# Autodesk Inventor assembly: ASM_Quarter_Piece_Assembly_Final
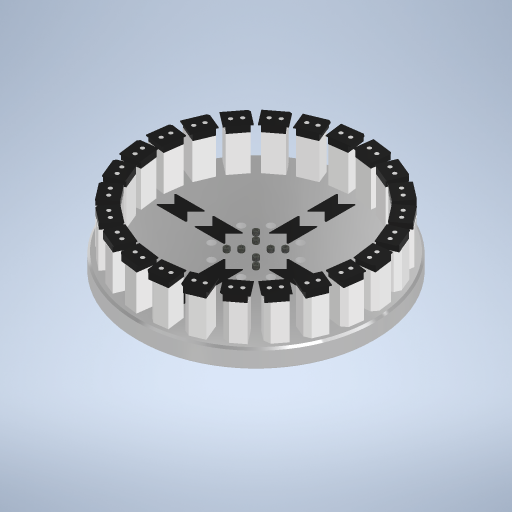
[picture p0: Inventor's stored thumbnail of the model, 512x512]
Saved by Autodesk Inventor 2024 (Build 280153000, 153)
## iProperties
Created: 2024-04-24
Part Number: ASM_Quarter_Piece_Assembly_Final
Document SubType Name: Assembly
Designer: jamha
Author: jamha
## Documents named in this file (6)
- C:\Users\jamha\OneDrive - The University of Texas at Dallas\SD - TEAM 1830\CAD\James\CAD Final Deliverable\ASM_Quarter_Piece_Assembly_Final.iam
- C:\Users\jamha\OneDrive - The University of Texas at Dallas\SD - TEAM 1830\CAD\James\CAD Final Deliverable\Quarter Sample Tray 8in Radius Final.ipt
- C:\Users\jamha\OneDrive - The University of Texas at Dallas\SD - TEAM 1830\CAD\James\CAD Final Deliverable\Dovetail Connecter.ipt
- C:\Users\jamha\OneDrive - The University of Texas at Dallas\SD - TEAM 1830\CAD\James\CAD Final Deliverable\ASM_Vial_and_Header.iam
- C:\Users\jamha\OneDrive - The University of Texas at Dallas\SD - TEAM 1830\CAD\James\CAD Final Deliverable\ASM_HDR50_Motor_and_ConnectorPlate.iam
- C:\Users\jamha\OneDrive - The University of Texas at Dallas\SD - TEAM 1830\CAD\James\CAD Final Deliverable\IPT_0.25_20 Screw.ipt
## Components (45 placed, 5 different names)
1. Quarter Sample Tray 8in Radius Final:1 — Mate:1, Flush:1, Flush:2, Mate:4, Mate:10, Mate:11
2. Quarter Sample Tray 8in Radius Final:2 — Mate:1, Flush:1, Flush:2, Mate:2, Flush:3, Mate:3, Flush:5, Mate:6, Angle:1, Mate:15, Mate:16
3. Quarter Sample Tray 8in Radius Final:3 — Mate:2, Flush:3, Mate:3, Mate:5, Flush:4, Flush:6, Mate:7, Mate:8, Mate:9, Mate:12, Mate:13, Mate:14
4. Quarter Sample Tray 8in Radius Final:4 — Mate:4, Mate:5, Flush:4
5. ASM_HDR50_Motor_and_ConnectorPlate:1 [sub-assembly] — Mate:10, Mate:11, Mate:12
6. Dovetail Connecter:2 — Flush:5, Mate:6
7. Dovetail Connecter:9
8. Dovetail Connecter:10
9. Dovetail Connecter:11
10. Dovetail Connecter:1 — Flush:6, Angle:1
11. Dovetail Connecter:12
12. Dovetail Connecter:13
13. Dovetail Connecter:14
14. ASM_Vial_and_Header:1 [sub-assembly] — Mate:7, Mate:8, Mate:9
15. ASM_Vial_and_Header:2 [sub-assembly]
16. ASM_Vial_and_Header:3 [sub-assembly]
17. ASM_Vial_and_Header:4 [sub-assembly]
18. ASM_Vial_and_Header:5 [sub-assembly]
19. ASM_Vial_and_Header:6 [sub-assembly]
20. ASM_Vial_and_Header:7 [sub-assembly]
21. ASM_Vial_and_Header:8 [sub-assembly]
22. ASM_Vial_and_Header:9 [sub-assembly]
23. ASM_Vial_and_Header:10 [sub-assembly]
24. ASM_Vial_and_Header:11 [sub-assembly]
25. ASM_Vial_and_Header:12 [sub-assembly]
26. ASM_Vial_and_Header:13 [sub-assembly]
27. ASM_Vial_and_Header:14 [sub-assembly]
28. ASM_Vial_and_Header:15 [sub-assembly]
29. ASM_Vial_and_Header:16 [sub-assembly]
30. ASM_Vial_and_Header:17 [sub-assembly]
31. ASM_Vial_and_Header:18 [sub-assembly]
32. ASM_Vial_and_Header:19 [sub-assembly]
33. ASM_Vial_and_Header:20 [sub-assembly]
34. ASM_Vial_and_Header:21 [sub-assembly]
35. ASM_Vial_and_Header:22 [sub-assembly]
36. ASM_Vial_and_Header:23 [sub-assembly]
37. ASM_Vial_and_Header:24 [sub-assembly]
38. 91251A543_Black-Oxide Alloy Steel Socket:1 — Mate:13, Mate:14
39. 91251A543_Black-Oxide Alloy Steel Socket:2
40. 91251A543_Black-Oxide Alloy Steel Socket:3
41. 91251A543_Black-Oxide Alloy Steel Socket:4
42. 91251A543_Black-Oxide Alloy Steel Socket:5 — Mate:15, Mate:16
43. 91251A543_Black-Oxide Alloy Steel Socket:6
44. 91251A543_Black-Oxide Alloy Steel Socket:7
45. 91251A543_Black-Oxide Alloy Steel Socket:8
## Component patterns: (4 elements, first: Dovetail Connecter:2), (4 elements, first: Dovetail Connecter:1), (24 elements, first: ASM_Vial_and_Header:1), (4 elements, first: 91251A543_Black-Oxide Alloy Steel Socket:1), (4 elements, first: 91251A543_Black-Oxide Alloy Steel Socket:5)
## Relationships (23: Mate 16, Flush 6, Angle 1)
- Mate:1: Quarter Sample Tray 8in Radius Final:1 ↔ Quarter Sample Tray 8in Radius Final:2
- Flush:1: Quarter Sample Tray 8in Radius Final:1 ↔ Quarter Sample Tray 8in Radius Final:2
- Flush:2: Quarter Sample Tray 8in Radius Final:1 ↔ Quarter Sample Tray 8in Radius Final:2
- Mate:2: Quarter Sample Tray 8in Radius Final:2 ↔ Quarter Sample Tray 8in Radius Final:3
- Flush:3: Quarter Sample Tray 8in Radius Final:2 ↔ Quarter Sample Tray 8in Radius Final:3
- Mate:3: Quarter Sample Tray 8in Radius Final:2 ↔ Quarter Sample Tray 8in Radius Final:3
- Mate:4: Quarter Sample Tray 8in Radius Final:1 ↔ Quarter Sample Tray 8in Radius Final:4
- Mate:5: Quarter Sample Tray 8in Radius Final:3 ↔ Quarter Sample Tray 8in Radius Final:4
- Flush:4: Quarter Sample Tray 8in Radius Final:3 ↔ Quarter Sample Tray 8in Radius Final:4
- Flush:5: Quarter Sample Tray 8in Radius Final:2 ↔ Dovetail Connecter:2
- Mate:6: Quarter Sample Tray 8in Radius Final:2 ↔ Dovetail Connecter:2
- Flush:6: Quarter Sample Tray 8in Radius Final:3 ↔ Dovetail Connecter:1
- Angle:1 (0 deg): Quarter Sample Tray 8in Radius Final:2 ↔ Dovetail Connecter:1
- Mate:7: Quarter Sample Tray 8in Radius Final:3 ↔ ASM_Vial_and_Header:1
- Mate:8: Quarter Sample Tray 8in Radius Final:3 ↔ ASM_Vial_and_Header:1
- Mate:9: Quarter Sample Tray 8in Radius Final:3 ↔ ASM_Vial_and_Header:1
- Mate:10: Quarter Sample Tray 8in Radius Final:1 ↔ ASM_HDR50_Motor_and_ConnectorPlate:1
- Mate:11: Quarter Sample Tray 8in Radius Final:1 ↔ ASM_HDR50_Motor_and_ConnectorPlate:1
- Mate:12: Quarter Sample Tray 8in Radius Final:3 ↔ ASM_HDR50_Motor_and_ConnectorPlate:1
- Mate:13: Quarter Sample Tray 8in Radius Final:3 ↔ 91251A543_Black-Oxide Alloy Steel Socket:1
- Mate:14: Quarter Sample Tray 8in Radius Final:3 ↔ 91251A543_Black-Oxide Alloy Steel Socket:1
- Mate:15: Quarter Sample Tray 8in Radius Final:2 ↔ 91251A543_Black-Oxide Alloy Steel Socket:5
- Mate:16: Quarter Sample Tray 8in Radius Final:2 ↔ 91251A543_Black-Oxide Alloy Steel Socket:5
